# Autodesk Inventor assembly: Robot
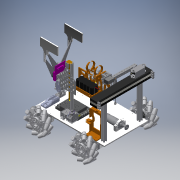
[picture p0: Inventor's stored thumbnail of the model, 180x180]
Saved by Autodesk Inventor 2017 (Build 210142000, 142)
## iProperties
Created: 2017-09-30
Part Number: Robot
Document SubType Name: Assembly
Designer: User
Author: User
## Documents named in this file (19)
- C:\Robotics\CAD\2017-18_CAD\Miscellaneous\Robot.iam
- C:\Robotics\CAD\2017-18_CAD\PlateFrame1.ipt
- C:\Robotics\CAD\2017-18_CAD\DirectDriveMotorSubAsembly.iam
- C:\Robotics\CAD\2017-18_CAD\batteryholder.ipt
- C:\Robotics\CAD\2017-18_CAD\Miscellaneous\JewlArm.iam
- C:\Robotics\CAD\2017-18_CAD\MotorProtector.ipt
- C:\Robotics\CAD\2017-18_CAD\Numbers.ipt
- C:\Robotics\CAD\2017-18_CAD\Phone_Cas.ipt
- C:\Robotics\CAD\2017-18_CAD\Miscellaneous\FlagHolder.ipt
- C:\Robotics\CAD\COTSParts\Rev\REV-31-1153RevHub.ipt
- C:\Robotics\CAD\COTSParts\Rev\REV-11-1144.ipt
- C:\Robotics\CAD\2017-18_CAD\Claw2017-18.iam
- C:\Robotics\CAD\COTSParts\Tetrix\tetrix-motor-mounts-1.snapshot.1\Tetrex 2pc motor mount.ipt
- C:\Robotics\CAD\COTSParts\Motors\Andymark 2964  NeveRest 40 Motor.ipt
- C:\Robotics\CAD\COTSParts\Actobotics\615 parts\615450.ipt
- C:\Robotics\CAD\2017-18_CAD\RelicArmLance.iam
- C:\Robotics\CAD\COTSParts\Bosch Extrusion\Bosch 20x20 8.5inch.ipt
- C:\Robotics\CAD\COTSParts\Tetrix\Tetrix Battery.ipt
- C:\Robotics\CAD\2017-18_CAD\Gen 1\Spacer.ipt
## Components (23 placed, 18 different names)
1. PlateFrame1:1 — Mate:1, Mate:2, Mate:3, Mate:4, Mate:6, Mate:7, Mate:8, Mate:11, Mate:12, Mate:14, Mate:15, Mate:16, Mate:17, Mate:26, Mate:39, Flush:18, Flush:19, Mate:45, Flush:23, Flush:26, Flush:49, Flush:52, Flush:53, Mate:52, Mate:56, Mate:57, Mate:58, Mate:59, Flush:54, Flush:55, Angle:1, Mate:60, Mate:61, Angle:2, Mate:62, Mate:63, Mate:64, Flush:56, Flush:57, Angle:3, Mate:65, Mate:66, Flush:58, Flush:59, Flush:60, Flush:61
2. DirectDriveMotorSubAsembly:1 [sub-assembly] — Mate:1, Mate:2, Mate:3
3. DirectDriveMotorSubAsembly:3 [sub-assembly] — Mate:11, Mate:12, Mate:17
4. DirectDriveMotorSubAsembly:2 [sub-assembly] — Mate:14, Mate:15, Mate:16, Insert:1
5. DirectDriveMotorSubAsembly:4 [sub-assembly] — Mate:4, Mate:6, Mate:7, Mate:8
6. batteryholder:1 — Mate:26, Flush:18, Flush:19, Mate:46, Mate:69, Mate:70, Mate:71
7. JewlArm:1 [sub-assembly] — Mate:39, Flush:26, Flush:49, Insert:4, Insert:5
8. MotorProtector:1 — Insert:1
9. Numbers:1 — Mate:45, Mate:46, Flush:23
10. Phone_Cas:1 — Flush:52, Flush:53, Mate:52
11. FlagHolder:1 — Mate:56
12. REV-31-1153RevHub:1 — Mate:57, Angle:1, Mate:60, Mate:61
13. REV-11-1144:1 — Mate:58, Angle:2, Mate:62, Mate:63
14. Claw2017-18:1 [sub-assembly] — Mate:59, Flush:54, Flush:55
15. Tetrex 2pc motor mount:1 — Mate:64, Flush:56, Insert:2
16. Andymark 2964  NeveRest 40 Motor:1 — Insert:2, Insert:3, Angle:3
17. 615450:1 — Insert:3, Flush:57
18. RelicArmLance:1 [sub-assembly] — Mate:68, Flush:61, Flush:62
19. Bosch 20x20 8.5inch:1 — Mate:66, Flush:58, Mate:67, Flush:62
20. Bosch 20x20 8.5inch:2 — Mate:65, Flush:59, Mate:67, Flush:60, Mate:68
21. Tetrix Battery:1 — Mate:69, Mate:70, Mate:71
22. Spacer:1 — Insert:4
23. Spacer:2 — Insert:5
## Relationships (58: Mate 34, Flush 16, Insert 5, Angle 3)
- Mate:1: PlateFrame1:1 ↔ DirectDriveMotorSubAsembly:1
- Mate:2: PlateFrame1:1 ↔ DirectDriveMotorSubAsembly:1
- Mate:3: PlateFrame1:1 ↔ DirectDriveMotorSubAsembly:1
- Mate:4: PlateFrame1:1 ↔ DirectDriveMotorSubAsembly:4
- Mate:6: PlateFrame1:1 ↔ DirectDriveMotorSubAsembly:4
- Mate:7: PlateFrame1:1 ↔ DirectDriveMotorSubAsembly:4
- Mate:8: PlateFrame1:1 ↔ DirectDriveMotorSubAsembly:4
- Mate:11: PlateFrame1:1 ↔ DirectDriveMotorSubAsembly:3
- Mate:12: PlateFrame1:1 ↔ DirectDriveMotorSubAsembly:3
- Mate:14: PlateFrame1:1 ↔ DirectDriveMotorSubAsembly:2
- Mate:15: PlateFrame1:1 ↔ DirectDriveMotorSubAsembly:2
- Mate:16: PlateFrame1:1 ↔ DirectDriveMotorSubAsembly:2
- Mate:17: PlateFrame1:1 ↔ DirectDriveMotorSubAsembly:3
- Mate:26: PlateFrame1:1 ↔ batteryholder:1
- Mate:39 (12.7 mm): PlateFrame1:1 ↔ JewlArm:1
- Flush:18 (1.5875 mm): PlateFrame1:1 ↔ batteryholder:1
- Flush:19 (19.05 mm): PlateFrame1:1 ↔ batteryholder:1
- Insert:1: DirectDriveMotorSubAsembly:2 ↔ MotorProtector:1
- Mate:45: PlateFrame1:1 ↔ Numbers:1
- Mate:46: batteryholder:1 ↔ Numbers:1
- Flush:23: PlateFrame1:1 ↔ Numbers:1
- Flush:26 (152.4 mm): PlateFrame1:1 ↔ JewlArm:1
- Flush:49: PlateFrame1:1 ↔ JewlArm:1
- Flush:52: PlateFrame1:1 ↔ Phone_Cas:1
- Flush:53 (50.8 mm): PlateFrame1:1 ↔ Phone_Cas:1
- Mate:52: PlateFrame1:1 ↔ Phone_Cas:1
- Mate:56: PlateFrame1:1 ↔ FlagHolder:1
- Mate:57: PlateFrame1:1 ↔ REV-31-1153RevHub:1
- Mate:58: PlateFrame1:1 ↔ REV-11-1144:1
- Mate:59: PlateFrame1:1 ↔ Claw2017-18:1
- Flush:54: PlateFrame1:1 ↔ Claw2017-18:1
- Flush:55 (-120.65 mm): PlateFrame1:1 ↔ Claw2017-18:1
- Angle:1 (270 deg): PlateFrame1:1 ↔ REV-31-1153RevHub:1
- Mate:60 (-76.2 mm): PlateFrame1:1 ↔ REV-31-1153RevHub:1
- Mate:61 (-50.8 mm): PlateFrame1:1 ↔ REV-31-1153RevHub:1
- Angle:2 (90 deg): PlateFrame1:1 ↔ REV-11-1144:1
- Mate:62 (-12.7 mm): PlateFrame1:1 ↔ REV-11-1144:1
- Mate:63 (-19.05 mm): PlateFrame1:1 ↔ REV-11-1144:1
- Mate:64: PlateFrame1:1 ↔ Tetrex 2pc motor mount:1
- Flush:56 (101.6 mm): PlateFrame1:1 ↔ Tetrex 2pc motor mount:1
- Insert:2: Tetrex 2pc motor mount:1 ↔ Andymark 2964  NeveRest 40 Motor:1
- Insert:3: Andymark 2964  NeveRest 40 Motor:1 ↔ 615450:1
- Flush:57: PlateFrame1:1 ↔ 615450:1
- Angle:3 (0 deg): PlateFrame1:1 ↔ Andymark 2964  NeveRest 40 Motor:1
- Mate:65: PlateFrame1:1 ↔ Bosch 20x20 8.5inch:2
- Mate:66: PlateFrame1:1 ↔ Bosch 20x20 8.5inch:1
- Flush:58 (19.05 mm): PlateFrame1:1 ↔ Bosch 20x20 8.5inch:1
- Flush:59 (19.05 mm): PlateFrame1:1 ↔ Bosch 20x20 8.5inch:2
- Mate:67 (209.55 mm): Bosch 20x20 8.5inch:1 ↔ Bosch 20x20 8.5inch:2
- Flush:60 (12.7 mm): PlateFrame1:1 ↔ Bosch 20x20 8.5inch:2
- Mate:68: RelicArmLance:1 ↔ Bosch 20x20 8.5inch:2
- Flush:61 (12.7 mm): PlateFrame1:1 ↔ RelicArmLance:1
- Flush:62 (-50.8 mm): RelicArmLance:1 ↔ Bosch 20x20 8.5inch:1
- Mate:69: batteryholder:1 ↔ Tetrix Battery:1
- Mate:70 (9.525 mm): batteryholder:1 ↔ Tetrix Battery:1
- Mate:71 (9.525 mm): batteryholder:1 ↔ Tetrix Battery:1
- Insert:4: JewlArm:1 ↔ Spacer:1
- Insert:5: JewlArm:1 ↔ Spacer:2
